# Autodesk Inventor assembly: Assembly1
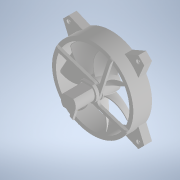
[picture p0: Inventor's stored thumbnail of the model, 180x180]
Saved by Autodesk Inventor 2021 (Build 250183000, 183)
## iProperties
Created: 2025-01-14
Part Number: Assembly1
Document SubType Name: Assembly
Designer: 24lucsil
Author: 24lucsil
## Documents named in this file (4)
- C:\Users\24lucsil\OneDrive - Hitachigymnasiet\Teknik\Wexteras\CAD\Assembly1.iam
- C:\Users\24lucsil\OneDrive - Hitachigymnasiet\Teknik\Wexteras\CAD\fläktFan.ipt
- C:\Users\24lucsil\OneDrive - Hitachigymnasiet\Teknik\Wexteras\CAD\FläktHållare.ipt
- C:\Users\24lucsil\OneDrive - Hitachigymnasiet\Teknik\Wexteras\CAD\FläktMotor.ipt
## Components (3 placed, 3 different names)
1. fläktFan:1 — Mate:1, Mate:2
2. FläktHållare:1
3. FläktMotor:1 — Mate:1, Mate:2
## Relationships (2: Mate 2)
- Mate:1: fläktFan:1 ↔ FläktMotor:1
- Mate:2 (4 mm): fläktFan:1 ↔ FläktMotor:1
